# Autodesk Inventor assembly: WG18and4SMAFeedthrough
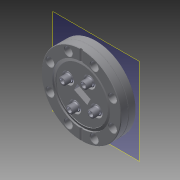
[picture p0: Inventor's stored thumbnail of the model, 180x180]
Saved by Autodesk Inventor 2015 (Build 190159000, 159)
## iProperties
Created: 2014-05-20
Part Number: WG18and4SMAFeedthrough
Document SubType Name: Assembly
Designer: jad211
Author: jad211
## Documents named in this file (3)
- C:\CADFiles\EDM Machine\EDM New Pumping Region\WG18and4SMAFeedthrough.iam
- C:\CADFiles\EDM Machine\EDM New Pumping Region\3-38sWithWG18Hole.ipt
- C:\CADFiles\Generic vacuum components\Imported Components\ifdcg012013\F0275X0501P_3.ipt
## Components (5 placed, 2 different names)
1. 3-38sWithWG18Hole:1 — Insert:1, Insert:2, Insert:3, Insert:4
2. F0275X0501P_3:1 — Insert:3
3. F0275X0501P_3:2 — Insert:2
4. F0275X0501P_3:3 — Insert:4
5. F0275X0501P_3:4 — Insert:1
## Relationships (4: Insert 4)
- Insert:1: 3-38sWithWG18Hole:1 ↔ F0275X0501P_3:4
- Insert:2: 3-38sWithWG18Hole:1 ↔ F0275X0501P_3:2
- Insert:3: 3-38sWithWG18Hole:1 ↔ F0275X0501P_3:1
- Insert:4: 3-38sWithWG18Hole:1 ↔ F0275X0501P_3:3
